# Autodesk Inventor assembly: motor
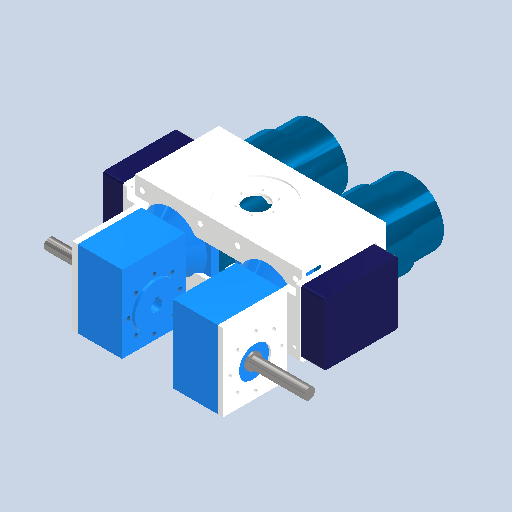
[picture p0: Inventor's stored thumbnail of the model, 512x512]
Saved by Autodesk Inventor 2025.3 (Build 293356030, 356C)
## iProperties
Created: 2025-09-06
Part Number: motor
Document SubType Name: Assembly
Designer: MSI
Mass: 13463.8 g
Surface Area: 5288.33 cm^2
Volume: 4261.47 cm^3
Density: 3.15942 g/cm^3
Author: MSI
## Documents named in this file (7)
- C:\Users\MSI\Desktop\Project\3. 로봇팔\Robot Arm Model\Robot_Arm_6_v1\motor.iam
- C:\Users\MSI\Desktop\Project\3. 로봇팔\Robot Arm Model\Robot_Arm_6_v1\NMRV30_motor.iam
- C:\Users\MSI\Desktop\Project\3. 로봇팔\Robot Arm Model\Robot_Arm_6_v1\motor_holder.ipt
- C:\Users\MSI\Desktop\Project\3. 로봇팔\Robot Arm Model\Robot_Arm_6_v1\motor_shaft.ipt
- C:\Users\MSI\Desktop\Project\3. 로봇팔\Robot Arm Model\Robot_Arm_6_v1\motor_driver.ipt
- C:\Users\MSI\Desktop\Project\3. 로봇팔\Robot Arm Model\Robot_Arm_6_v1\motor_driver_frame_r.ipt
- C:\Users\MSI\Desktop\Project\3. 로봇팔\Robot Arm Model\Robot_Arm_6_v1\motor_driver_frame_l.ipt
## Components (10 placed, 6 different names)
1. NMRV30_motor:1 [sub-assembly] — 강체:1, 강체:3, 회전:2, 강체:8
2. NMRV30_motor:2 [sub-assembly] — 강체:2, 강체:4, 회전:1, 강체:9
3. motor_holder:1 — 강체:1, 강체:2
4. motor_holder:2 — 강체:3, 강체:4
5. motor_shaft:1 — 회전:1
6. motor_shaft:2 — 회전:2
7. motor_driver:1 — 강체:6
8. motor_driver:2 — 강체:7
9. motor_driver_frame_r:1 — 강체:8, 강체:7
10. motor_driver_frame_l:1 — 강체:9, 강체:6
## Relationships (10: WeldJoint 8, RevoluteJoint 2)
- 강체:1 [WeldJoint]: NMRV30_motor:1 ↔ motor_holder:1
- 강체:2 [WeldJoint]: NMRV30_motor:2 ↔ motor_holder:1
- 강체:3 [WeldJoint]: NMRV30_motor:1 ↔ motor_holder:2
- 강체:4 [WeldJoint]: NMRV30_motor:2 ↔ motor_holder:2
- 회전:1 [RevoluteJoint]: NMRV30_motor:2 ↔ motor_shaft:1
- 회전:2 [RevoluteJoint]: NMRV30_motor:1 ↔ motor_shaft:2
- 강체:6 [WeldJoint]: motor_driver:1 ↔ motor_driver_frame_l:1
- 강체:7 [WeldJoint]: motor_driver:2 ↔ motor_driver_frame_r:1
- 강체:8 [WeldJoint]: NMRV30_motor:1 ↔ motor_driver_frame_r:1
- 강체:9 [WeldJoint]: NMRV30_motor:2 ↔ motor_driver_frame_l:1
